# Autodesk Inventor assembly: CAR_023_KickerAssembly
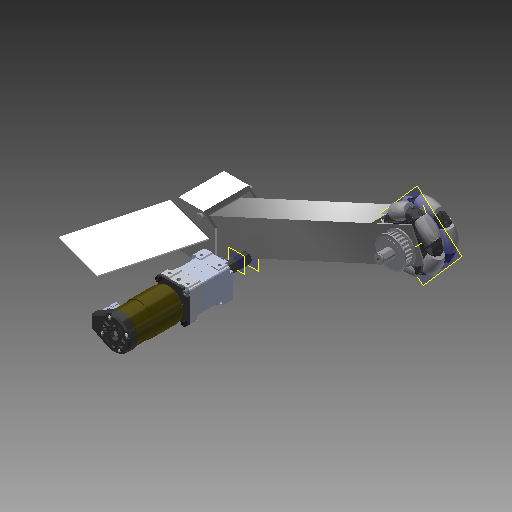
[picture p0: Inventor's stored thumbnail of the model, 512x512]
Saved by Autodesk Inventor 2018 (Build 220112000, 112)
## iProperties
Created: 2020-02-02
Part Number: CAR_023_KickerAssembly
Document SubType Name: Assembly
Designer: user
Author: user
## Documents named in this file (10)
- C:\Users\Sam\Desktop\GrabCad\Infinite Recharge 2020\Build season\CAR_023_KickerAssembly.iam
- C:\Users\Sam\Desktop\GrabCad\Infinite Recharge 2020\Build season\3 inch OmniWheel STEP\3_25_Omni-Directional_Wheel_217-4775.iam
- C:\Users\Sam\Desktop\GrabCad\Infinite Recharge 2020\Build season\CAR_024_KickerUChannel.ipt
- C:\Users\Sam\Desktop\GrabCad\Infinite Recharge 2020\Build season\CAR_025_KickerBar.ipt
- C:\Users\Sam\Desktop\GrabCad\Infinite Recharge 2020\Brainstorming\Versaplanetary\Versa+Motor.iam
- C:\Users\Sam\Desktop\GrabCad\Infinite Recharge 2020\Build season\DGB STEP\217-4006_0_500_flanged_thunderhex_bearing.ipt
- C:\Users\Sam\Desktop\GrabCad\Infinite Recharge 2020\Build season\CAR_028_98306A173_STEEL CLEVIS PIN.ipt
- C:\Users\Sam\Desktop\GrabCad\Infinite Recharge 2020\Build season\CAR_029_KickerAxle.ipt
- C:\Users\Sam\Desktop\GrabCad\Infinite Recharge 2020\Build season\CAR_030_24t_x_9mm_Wide_Double_Flange_Aluminum_Pulley_HTD_5mm_1_2_Hex_Bore_217-3227.ipt
- C:\Users\Sam\Desktop\GrabCad\Infinite Recharge 2020\Build season\CAR_031_VersaplanetaryMountPlate.ipt
## Components (12 placed, 9 different names)
1. 3_25_Omni-Directional_Wheel_217-4775:1 [sub-assembly] — Mate:5, Mate:9
2. CAR_024_KickerUChannel:1 — Mate:1, Mate:2, Insert:1, Insert:2, Insert:3, Flush:1, Mate:15, Angle:1
3. CAR_025_KickerBar:1 — Mate:1, Mate:2, Mate:5, Mate:6, Mate:7, Mate:10, Mate:11, Tangent:1
4. Versa+Motor:1 [sub-assembly] — Mate:16, Angle:2
5. 217-4006_0_500_flanged_thunderhex_bearing:1 — Mate:6, Mate:8, Mate:11, Mate:14
6. 217-4006_0_500_flanged_thunderhex_bearing:2 — Mate:7, Mate:8, Mate:9, Mate:10, Insert:4
7. CAR_028_98306A173_STEEL CLEVIS PIN:1 — Insert:2, Tangent:1
8. CAR_028_98306A173_STEEL CLEVIS PIN:2 — Insert:3
9. CAR_028_98306A173_STEEL CLEVIS PIN:3 — Insert:1
10. CAR_029_KickerAxle:1 — Mate:12, Mate:13, Insert:4
11. CAR_030_24t_x_9mm_Wide_Double_Flange_Aluminum_Pulley_HTD_5mm_1_2_Hex_Bore_217-3227:1 — Mate:12, Mate:13, Mate:14
12. CAR_031_VersaplanetaryMountPlate:1 — Flush:1, Mate:15, Angle:1, Mate:16, Angle:2
## Relationships (22: Mate 14, Insert 4, Angle 2, Tangent 1, Flush 1)
- Mate:1: CAR_024_KickerUChannel:1 ↔ CAR_025_KickerBar:1
- Mate:2: CAR_024_KickerUChannel:1 ↔ CAR_025_KickerBar:1
- Mate:5: 3_25_Omni-Directional_Wheel_217-4775:1 ↔ CAR_025_KickerBar:1
- Mate:6 (-20.6375 mm): CAR_025_KickerBar:1 ↔ 217-4006_0_500_flanged_thunderhex_bearing:1
- Mate:7: CAR_025_KickerBar:1 ↔ 217-4006_0_500_flanged_thunderhex_bearing:2
- Mate:8: 217-4006_0_500_flanged_thunderhex_bearing:1 ↔ 217-4006_0_500_flanged_thunderhex_bearing:2
- Mate:9: 3_25_Omni-Directional_Wheel_217-4775:1 ↔ 217-4006_0_500_flanged_thunderhex_bearing:2
- Mate:10: CAR_025_KickerBar:1 ↔ 217-4006_0_500_flanged_thunderhex_bearing:2
- Mate:11: CAR_025_KickerBar:1 ↔ 217-4006_0_500_flanged_thunderhex_bearing:1
- Insert:1: CAR_024_KickerUChannel:1 ↔ CAR_028_98306A173_STEEL CLEVIS PIN:3
- Insert:2: CAR_024_KickerUChannel:1 ↔ CAR_028_98306A173_STEEL CLEVIS PIN:1
- Insert:3: CAR_024_KickerUChannel:1 ↔ CAR_028_98306A173_STEEL CLEVIS PIN:2
- Mate:12: CAR_029_KickerAxle:1 ↔ CAR_030_24t_x_9mm_Wide_Double_Flange_Aluminum_Pulley_HTD_5mm_1_2_Hex_Bore_217-3227:1
- Mate:13: CAR_029_KickerAxle:1 ↔ CAR_030_24t_x_9mm_Wide_Double_Flange_Aluminum_Pulley_HTD_5mm_1_2_Hex_Bore_217-3227:1
- Mate:14: 217-4006_0_500_flanged_thunderhex_bearing:1 ↔ CAR_030_24t_x_9mm_Wide_Double_Flange_Aluminum_Pulley_HTD_5mm_1_2_Hex_Bore_217-3227:1
- Tangent:1: CAR_025_KickerBar:1 ↔ CAR_028_98306A173_STEEL CLEVIS PIN:1
- Insert:4 (-2.3368 mm): 217-4006_0_500_flanged_thunderhex_bearing:2 ↔ CAR_029_KickerAxle:1
- Flush:1: CAR_024_KickerUChannel:1 ↔ CAR_031_VersaplanetaryMountPlate:1
- Mate:15: CAR_024_KickerUChannel:1 ↔ CAR_031_VersaplanetaryMountPlate:1
- Angle:1 (15 deg): CAR_024_KickerUChannel:1 ↔ CAR_031_VersaplanetaryMountPlate:1
- Mate:16: Versa+Motor:1 ↔ CAR_031_VersaplanetaryMountPlate:1
- Angle:2 (-15 deg): Versa+Motor:1 ↔ CAR_031_VersaplanetaryMountPlate:1
